# Autodesk Inventor assembly: Idler Sprocket 16t
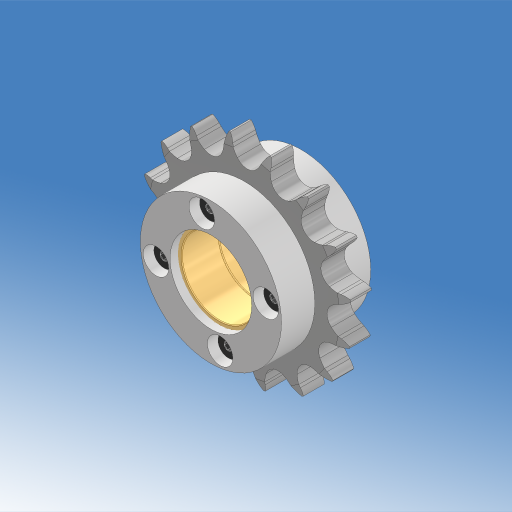
[picture p0: Inventor's stored thumbnail of the model, 512x512]
Saved by Autodesk Inventor 2024 (Build 280153000, 153)
## iProperties
Created: 2023-01-21
Part Number: Idler Sprocket 16t
Document SubType Name: Assembly
Designer: AdminForWorker
Title: Idler Sprocket 16t v12
Author: AdminForWorker
## Documents named in this file (6)
- C:\Users\seene\OneDrive\SBRT\Robocup Rescue\Drive\v1\TANK flipper\Idler Sprocket 16t v12.iam
- C:\Users\seene\OneDrive\SBRT\Robocup Rescue\Drive\v1\TANK flipper\2868T199_High-Load Oil-Embedded 863 Sleeve Bearing (1) v2.ipt
- C:\Users\seene\OneDrive\SBRT\Robocup Rescue\Drive\v1\TANK flipper\91259A166_Alloy Steel Shoulder Screw v2.ipt
- C:\Users\seene\OneDrive\SBRT\Robocup Rescue\Drive\v1\TANK flipper\Sprocket_.ipt
- C:\Users\seene\OneDrive\SBRT\Robocup Rescue\Drive\v1\TANK flipper\Part16.ipt
- C:\Users\seene\OneDrive\SBRT\Robocup Rescue\Drive\v1\TANK flipper\counterbore side.ipt
## Components (9 placed, 5 different names)
1. 2868T199_High-Load Oil-Embedded 863 Sleeve Bearing (1) v2:1 — Rigid:1
2. 2868T199_High-Load Oil-Embedded 863 Sleeve Bearing (1) v2:2 — Rigid:2
3. 91259A166_Alloy Steel Shoulder Screw v2:1 — Rigid:3
4. 91259A166_Alloy Steel Shoulder Screw v2:2 — Rotational:2
5. 91259A166_Alloy Steel Shoulder Screw v2:3 — Rigid:4
6. 91259A166_Alloy Steel Shoulder Screw v2:4 — Rotational:1
7. Sprocket\:1 — Mate:1, Mate:2, Mate:3, Mate:4, Mate:5, Rigid:1, Rigid:2, Rigid:3, Rigid:4, Rotational:1, Rotational:2
8. idler_spacer_inside — Mate:3, Mate:4, Mate:5
9. idler_spacer_outside — Mate:1, Mate:2
## Relationships (11: Mate 5, WeldJoint 4, RevoluteJoint 2)
- Mate:1: Sprocket\:1 ↔ idler_spacer_outside
- Mate:2: Sprocket\:1 ↔ idler_spacer_outside
- Mate:3: Sprocket\:1 ↔ idler_spacer_inside
- Mate:4: Sprocket\:1 ↔ idler_spacer_inside
- Mate:5: Sprocket\:1 ↔ idler_spacer_inside
- Rigid:1 [WeldJoint]: 2868T199_High-Load Oil-Embedded 863 Sleeve Bearing (1) v2:1 ↔ Sprocket\:1
- Rigid:2 [WeldJoint]: 2868T199_High-Load Oil-Embedded 863 Sleeve Bearing (1) v2:2 ↔ Sprocket\:1
- Rigid:3 [WeldJoint]: 91259A166_Alloy Steel Shoulder Screw v2:1 ↔ Sprocket\:1
- Rigid:4 [WeldJoint]: 91259A166_Alloy Steel Shoulder Screw v2:3 ↔ Sprocket\:1
- Rotational:1 [RevoluteJoint]: 91259A166_Alloy Steel Shoulder Screw v2:4 ↔ Sprocket\:1
- Rotational:2 [RevoluteJoint]: 91259A166_Alloy Steel Shoulder Screw v2:2 ↔ Sprocket\:1
